# Autodesk Inventor assembly: 射出_モーター
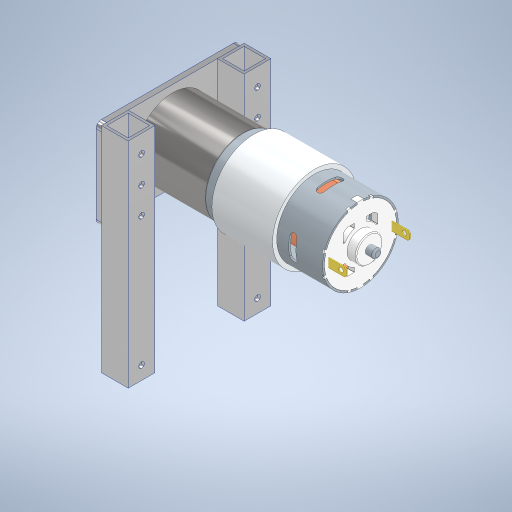
[picture p0: Inventor's stored thumbnail of the model, 512x512]
Saved by Autodesk Inventor 2023 (Build 270158000, 158)
## iProperties
Created: 2022-04-24
Part Number: 射出_モーター
Document SubType Name: Assembly
Designer: yuta
Author: yuta
## Documents named in this file (4)
- C:\Users\yuta\Documents\NHK\射出_モーター.iam
- C:\Users\yuta\Documents\NHK\射出_角柱1.ipt
- C:\Users\yuta\Documents\NHK\射出_モーター固定1.ipt
- C:\Users\yuta\Documents\NHK\RS775+gennsoku.iam
## Components (4 placed, 3 different names)
1. 射出_角柱1:2 — メイト:5, メイト:6, メイト:7, メイト:8
2. 射出_角柱1:3 — メイト:1, メイト:2, メイト:3, メイト:4
3. 射出_モーター固定1:1 — メイト:1, メイト:2, メイト:3, メイト:4, メイト:5, メイト:6, メイト:7, メイト:8, メイト:9, メイト:10
4. RS775+gennsoku:1 [sub-assembly] — メイト:9, メイト:10
## Relationships (10: Mate 10)
- メイト:1 [Mate]: 射出_角柱1:3 ↔ 射出_モーター固定1:1
- メイト:2 [Mate]: 射出_角柱1:3 ↔ 射出_モーター固定1:1
- メイト:3 [Mate]: 射出_角柱1:3 ↔ 射出_モーター固定1:1
- メイト:4 [Mate]: 射出_角柱1:3 ↔ 射出_モーター固定1:1
- メイト:5 [Mate]: 射出_角柱1:2 ↔ 射出_モーター固定1:1
- メイト:6 [Mate]: 射出_角柱1:2 ↔ 射出_モーター固定1:1
- メイト:7 [Mate]: 射出_角柱1:2 ↔ 射出_モーター固定1:1
- メイト:8 [Mate]: 射出_角柱1:2 ↔ 射出_モーター固定1:1
- メイト:9 [Mate]: 射出_モーター固定1:1 ↔ RS775+gennsoku:1
- メイト:10 [Mate]: 射出_モーター固定1:1 ↔ RS775+gennsoku:1
